# Autodesk Inventor assembly: birdeye_wristUnit
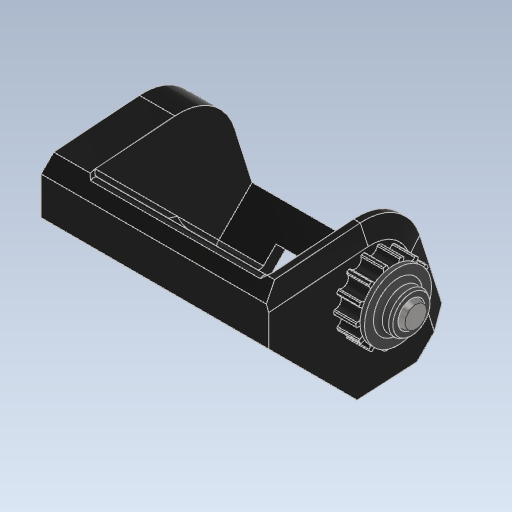
[picture p0: Inventor's stored thumbnail of the model, 512x512]
Saved by Autodesk Inventor 2024 (Build 280153000, 153)
## iProperties
Created: 2023-09-25
Part Number: birdeye_wristUnit
Document SubType Name: Assembly
Designer: michi
Author: michi
## Documents named in this file (4)
- C:\Users\michi\OneDrive - Kyoto University\lab\6_SHINOBI\FUHGA4\Design_Mechanism\05_birdeye\birdeye_wristUnit.iam
- C:\Users\michi\OneDrive - Kyoto University\lab\6_SHINOBI\FUHGA4\Design_Mechanism\05_birdeye\birdeye_wristUnit\brideye_wristUnit_pully_passive_withCameraMouter.ipt
- C:\Users\michi\OneDrive - Kyoto University\lab\6_SHINOBI\FUHGA4\Design_Mechanism\05_birdeye\birdeye_wristUnit\_MS3-6.ipt
- C:\Users\michi\OneDrive - Kyoto University\lab\6_SHINOBI\FUHGA4\Design_Mechanism\05_birdeye\birdeye_wristUnit\_GFM-0304-02.ipt
## Components (5 placed, 3 different names)
1. brideye_wristUnit_pully_passive_withCameraMouter:1 — メイト:1, メイト:2, 正接:1, 正接:2, 回転:1, 回転:2
2. _MS3-6:1 — メイト:1, 正接:1
3. _MS3-6:2 — メイト:2, 正接:2
4. _GFM-0304-02:2 — 回転:1
5. _GFM-0304-02:3 — 回転:2
## Relationships (6: Mate 2, Tangent 2, RevoluteJoint 2)
- メイト:1 [Mate]: brideye_wristUnit_pully_passive_withCameraMouter:1 ↔ _MS3-6:1
- メイト:2 [Mate]: brideye_wristUnit_pully_passive_withCameraMouter:1 ↔ _MS3-6:2
- 正接:1 [Tangent]: brideye_wristUnit_pully_passive_withCameraMouter:1 ↔ _MS3-6:1
- 正接:2 [Tangent]: brideye_wristUnit_pully_passive_withCameraMouter:1 ↔ _MS3-6:2
- 回転:1 [RevoluteJoint]: brideye_wristUnit_pully_passive_withCameraMouter:1 ↔ _GFM-0304-02:2
- 回転:2 [RevoluteJoint]: brideye_wristUnit_pully_passive_withCameraMouter:1 ↔ _GFM-0304-02:3
